# Autodesk Inventor assembly: CL7-200
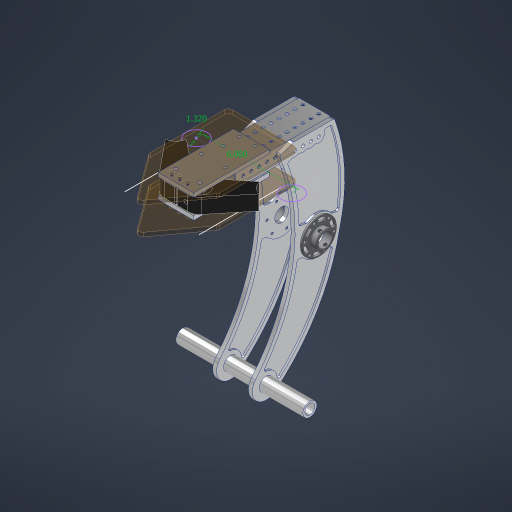
[picture p0: Inventor's stored thumbnail of the model, 512x512]
Saved by Autodesk Inventor 2023.4 (Build 274418000, 418)
## iProperties
Created: 2025-03-17
Part Number: CL7-200
Document SubType Name: Assembly
Designer: dlangdon
Author: dlangdon
## Documents named in this file (9)
- C:\Users\brand\OneDrive\Documents\GitHub\robotics 23\2025-ReefScape---CAD\Climber\CL7\CL7-200.iam
- C:\Users\brand\OneDrive\Documents\GitHub\robotics 23\2025-ReefScape---CAD\Climber\CL7\CL7-005.ipt
- C:\Users\brand\OneDrive\Documents\GitHub\robotics 23\2025-ReefScape---CAD\Climber\CL7\CL7-004.ipt
- C:\Users\brand\OneDrive\Documents\GitHub\robotics 23\2025-ReefScape---CAD\Climber\CL7\CL7-005aa.ipt
- C:\Users\brand\OneDrive\Documents\GitHub\robotics 23\2025-ReefScape---CAD\Climber\CL7\CL7-006.ipt
- C:\Users\brand\OneDrive\Documents\GitHub\robotics 23\2025-ReefScape---CAD\Climber\CL7\CL7-008.ipt
- C:\Users\brand\OneDrive\Documents\GitHub\robotics 23\2025-ReefScape---CAD\Climber\CL7\CL7-009.ipt
- C:\Users\brand\OneDrive\Documents\GitHub\robotics 23\2025-ReefScape---CAD\Climber\CL7\CL-GB\CL7-GB-005.ipt
- C:\Users\brand\OneDrive\Documents\GitHub\robotics 23\2025-ReefScape---CAD\Climber\CL7\CL7-017.ipt
## Components (12 placed, 8 different names)
1. CL7-005:1 — Mate:4, Mate:5, Mate:6, Mate:7, Mate:8, Mate:9, Insert:1, Insert:2, Insert:13, Insert:14
2. CL7-004:1 — Mate:5, Flush:1, Symmetry:2, Flush:2
3. CL7-004:2 — Mate:4, Mate:6, Flush:1, Symmetry:2, Flush:2
4. CL7-005aa:1 — Mate:7, Mate:8, Mate:9, Insert:15, Insert:16
5. CL7-006:1 — Insert:1, Insert:2, Insert:3, Insert:4, Insert:5, Insert:6, Insert:7, Insert:8
6. CL7-008:1 — Insert:3, Insert:4, Symmetry:1, Insert:8, Insert:11, Insert:12
7. CL7-008:2 — Insert:5, Insert:6, Symmetry:1, Mate:10, Insert:7, Insert:9, Insert:10
8. CL7-009:1 — Mate:10, Mate:11
9. CL7-GB-005:1 — Insert:11, Insert:12
10. CL7-GB-005:2 — Insert:9, Insert:10
11. CL7-017:1 — Insert:13, Insert:14
12. CL7-017:2 — Insert:15, Insert:16
## Relationships (28: Insert 16, Mate 8, Flush 2, Symmetry 2)
- Mate:4: CL7-005:1 ↔ CL7-004:2
- Mate:5: CL7-005:1 ↔ CL7-004:1
- Mate:6 (0.7937 mm): CL7-005:1 ↔ CL7-004:2
- Flush:1: CL7-004:1 ↔ CL7-004:2
- Mate:7: CL7-005:1 ↔ CL7-005aa:1
- Mate:8: CL7-005:1 ↔ CL7-005aa:1
- Mate:9 (25.4 mm): CL7-005:1 ↔ CL7-005aa:1
- Insert:1: CL7-005:1 ↔ CL7-006:1
- Insert:2: CL7-005:1 ↔ CL7-006:1
- Insert:3: CL7-006:1 ↔ CL7-008:1
- Insert:4: CL7-006:1 ↔ CL7-008:1
- Insert:5: CL7-006:1 ↔ CL7-008:2
- Insert:6: CL7-006:1 ↔ CL7-008:2
- Symmetry:1: CL7-008:1 ↔ CL7-008:2
- Mate:10: CL7-008:2 ↔ CL7-009:1
- Mate:11: CL7-009:1
- Insert:7: CL7-006:1 ↔ CL7-008:2
- Insert:8: CL7-006:1 ↔ CL7-008:1
- Symmetry:2: CL7-004:1 ↔ CL7-004:2
- Flush:2: CL7-004:1 ↔ CL7-004:2
- Insert:9: CL7-008:2 ↔ CL7-GB-005:2
- Insert:10: CL7-008:2 ↔ CL7-GB-005:2
- Insert:11: CL7-008:1 ↔ CL7-GB-005:1
- Insert:12: CL7-008:1 ↔ CL7-GB-005:1
- Insert:13: CL7-005:1 ↔ CL7-017:1
- Insert:14: CL7-005:1 ↔ CL7-017:1
- Insert:15: CL7-005aa:1 ↔ CL7-017:2
- Insert:16: CL7-005aa:1 ↔ CL7-017:2
